# Autodesk Inventor assembly: raspberry_test
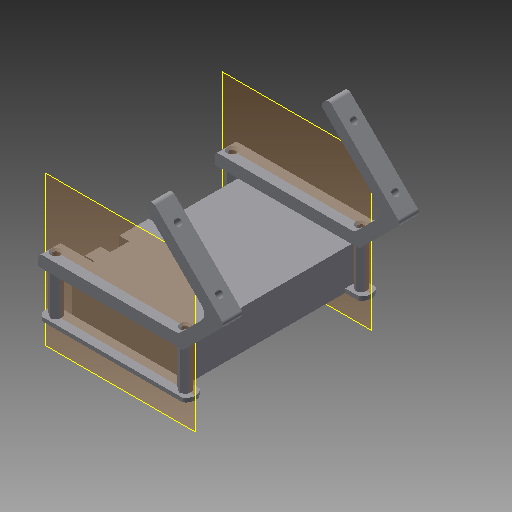
[picture p0: Inventor's stored thumbnail of the model, 512x512]
Saved by Autodesk Inventor 2019 (Build 230136000, 136)
## iProperties
Created: 2021-11-18
Part Number: raspberry_test
Document SubType Name: Assembly
Designer: Pokick
Author: Pokick
## Documents named in this file (3)
- C:\Users\Pokick\Desktop\PWR\SEM7\INZYNIER\maszyna\raspberry_test.iam
- C:\Users\Pokick\Desktop\PWR\SEM7\INZYNIER\maszyna\raspberry+touch.ipt
- C:\Users\Pokick\Desktop\PWR\SEM7\INZYNIER\maszyna\Part5.ipt
## Components (3 placed, 3 different names)
1. raspberry+touch:1 — Flush:1, Rotational:1
2. Raspberry_holder — Flush:1
3. Part5:2 — Rotational:1
## Relationships (2: Flush 1, RevoluteJoint 1)
- Flush:1: raspberry+touch:1 ↔ Raspberry_holder
- Rotational:1 [RevoluteJoint]: raspberry+touch:1 ↔ Part5:2
